# Autodesk Inventor assembly: fictief_zonnepaneel
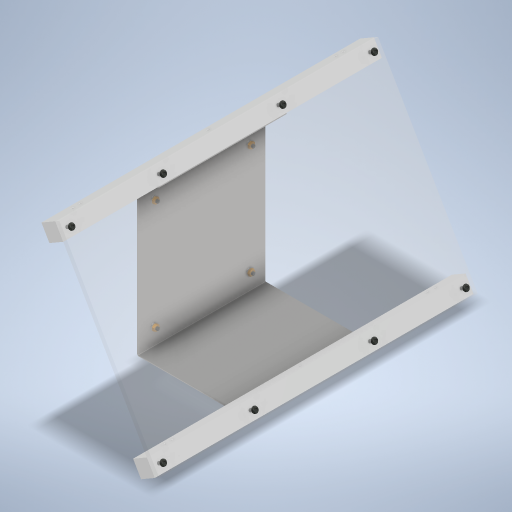
[picture p0: Inventor's stored thumbnail of the model, 512x512]
Saved by Autodesk Inventor 2023 (Build 270158000, 158)
## iProperties
Created: 2022-09-12
Part Number: fictief_zonnepaneel
Document SubType Name: Assembly
Designer: VoorL
Author: VoorL
## Documents named in this file (9)
- C:\Users\Ayoub\Documents\GitHub\zonnepaneel-concept\Opstelling_Zonnepaneel\fictief_zonnepaneel.iam
- C:\Users\Ayoub\Documents\GitHub\zonnepaneel-concept\Opstelling_Zonnepaneel\aluminium_stafmateriaal.ipt
- C:\Users\Ayoub\Documents\GitHub\zonnepaneel-concept\Opstelling_Zonnepaneel\Perspex_plaat.ipt
- C:\Users\Ayoub\Documents\GitHub\zonnepaneel-concept\Opstelling_Zonnepaneel\zetdeel_hoog.ipt
- C:\Users\Ayoub\Documents\GitHub\zonnepaneel-concept\Opstelling_Zonnepaneel\A4.ipt
- C:\Users\Ayoub\Documents\GitHub\zonnepaneel-concept\Opstelling_Zonnepaneel\rubberen_voetje.ipt
- C:\Users\Ayoub\Documents\GitHub\zonnepaneel-concept\Opstelling_Zonnepaneel\ISO 7380-1 - M4 x 10.ipt
- C:\Users\Ayoub\Documents\GitHub\zonnepaneel-concept\Opstelling_Zonnepaneel\DIN 125 - A 4,3.ipt
- C:\Users\Ayoub\Documents\GitHub\zonnepaneel-concept\Opstelling_Zonnepaneel\DIN EN ISO 4032 - M4.ipt
## Components (32 placed, 8 different names)
1. aluminium_stafmateriaal:1 — Mate:1, Mate:2, Mate:3
2. Perspex_plaat:1 — Mate:1, Mate:2, Mate:3, Mate:4, Mate:5, Mate:6, Mate:11, Flush:1, Flush:2, Insert:1, Insert:2, Insert:3, Insert:4, Insert:5, Insert:6, Insert:7, Insert:8
3. aluminium_stafmateriaal:2 — Mate:4, Mate:5, Mate:6, Mate:7, Mate:8, Mate:9
4. zetdeel_hoog:1 — Mate:7, Mate:8, Mate:9, Mate:10, Mate:12, Mate:13, Mate:14, Mate:15, Mate:16, Mate:17, Mate:18, Mate:19, Mate:26, Mate:27, Mate:29, Mate:31, Mate:32, Mate:33, Insert:10, Insert:11, Insert:12
5. A4:1 — Mate:11, Flush:1, Flush:2
6. rubberen_voetje:1 — Mate:12, Mate:16, Mate:20, Mate:21
7. rubberen_voetje:2 — Mate:15, Mate:19, Mate:24, Mate:25
8. rubberen_voetje:3 — Mate:13, Mate:17, Insert:9
9. rubberen_voetje:4 — Mate:14, Mate:18, Mate:22, Mate:23
10. ISO 7380-1 M4 x 10:1 — Insert:1
11. ISO 7380-1 M4 x 10:2 — Insert:2
12. ISO 7380-1 M4 x 10:3 — Insert:3
13. ISO 7380-1 M4 x 10:4 — Insert:4
14. ISO 7380-1 M4 x 10:5 — Insert:5
15. ISO 7380-1 M4 x 10:6 — Insert:6
16. ISO 7380-1 M4 x 10:7 — Insert:7
17. ISO 7380-1 M4 x 10:8 — Insert:8
18. ISO 7380-1 M4 x 10:9 — Insert:9, Mate:28, Mate:36
19. ISO 7380-1 M4 x 10:10 — Mate:20, Mate:21, Mate:34, Mate:41
20. ISO 7380-1 M4 x 10:11 — Mate:24, Mate:25, Mate:35, Mate:43
21. ISO 7380-1 M4 x 10:12 — Mate:22, Mate:23, Mate:30, Mate:38
22. DIN 125-1 A A 4,3:1 — Mate:28, Mate:29, Mate:37
23. DIN 125-1 A A 4,3:2 — Mate:32, Mate:35, Mate:42
24. DIN 125-1 A A 4,3:3 — Mate:33, Mate:34, Mate:40
25. DIN 125-1 A A 4,3:4 — Mate:30, Mate:31, Mate:39
26. DIN EN ISO 4032 M4:1 — Mate:36, Mate:37
27. DIN EN ISO 4032 M4:2 — Mate:38, Mate:39
28. DIN EN ISO 4032 M4:3 — Mate:40, Mate:41
29. DIN EN ISO 4032 M4:4 — Mate:42, Mate:43
30. ISO 7380-1 M4 x 10:13 — Insert:10
31. ISO 7380-1 M4 x 10:14 — Insert:11
32. ISO 7380-1 M4 x 10:15 — Insert:12
## Relationships (57: Mate 43, Insert 12, Flush 2)
- Mate:1: aluminium_stafmateriaal:1 ↔ Perspex_plaat:1
- Mate:2: aluminium_stafmateriaal:1 ↔ Perspex_plaat:1
- Mate:3: aluminium_stafmateriaal:1 ↔ Perspex_plaat:1
- Mate:4: Perspex_plaat:1 ↔ aluminium_stafmateriaal:2
- Mate:5: Perspex_plaat:1 ↔ aluminium_stafmateriaal:2
- Mate:6: Perspex_plaat:1 ↔ aluminium_stafmateriaal:2
- Mate:7: aluminium_stafmateriaal:2 ↔ zetdeel_hoog:1
- Mate:8: aluminium_stafmateriaal:2 ↔ zetdeel_hoog:1
- Mate:9: aluminium_stafmateriaal:2 ↔ zetdeel_hoog:1
- Mate:10: zetdeel_hoog:1
- Mate:11: Perspex_plaat:1 ↔ A4:1
- Flush:1 (50 mm): Perspex_plaat:1 ↔ A4:1
- Flush:2 (20 mm): Perspex_plaat:1 ↔ A4:1
- Mate:12: zetdeel_hoog:1 ↔ rubberen_voetje:1
- Mate:13: zetdeel_hoog:1 ↔ rubberen_voetje:3
- Mate:14: zetdeel_hoog:1 ↔ rubberen_voetje:4
- Mate:15: zetdeel_hoog:1 ↔ rubberen_voetje:2
- Mate:16: zetdeel_hoog:1 ↔ rubberen_voetje:1
- Mate:17: zetdeel_hoog:1 ↔ rubberen_voetje:3
- Mate:18: zetdeel_hoog:1 ↔ rubberen_voetje:4
- Mate:19: zetdeel_hoog:1 ↔ rubberen_voetje:2
- Insert:1: Perspex_plaat:1 ↔ ISO 7380-1 M4 x 10:1
- Insert:2: Perspex_plaat:1 ↔ ISO 7380-1 M4 x 10:2
- Insert:3: Perspex_plaat:1 ↔ ISO 7380-1 M4 x 10:3
- Insert:4: Perspex_plaat:1 ↔ ISO 7380-1 M4 x 10:4
- Insert:5: Perspex_plaat:1 ↔ ISO 7380-1 M4 x 10:5
- Insert:6: Perspex_plaat:1 ↔ ISO 7380-1 M4 x 10:6
- Insert:7: Perspex_plaat:1 ↔ ISO 7380-1 M4 x 10:7
- Insert:8: Perspex_plaat:1 ↔ ISO 7380-1 M4 x 10:8
- Insert:9: rubberen_voetje:3 ↔ ISO 7380-1 M4 x 10:9
- Mate:20: rubberen_voetje:1 ↔ ISO 7380-1 M4 x 10:10
- Mate:21: rubberen_voetje:1 ↔ ISO 7380-1 M4 x 10:10
- Mate:22: rubberen_voetje:4 ↔ ISO 7380-1 M4 x 10:12
- Mate:23: rubberen_voetje:4 ↔ ISO 7380-1 M4 x 10:12
- Mate:24: rubberen_voetje:2 ↔ ISO 7380-1 M4 x 10:11
- Mate:25: rubberen_voetje:2 ↔ ISO 7380-1 M4 x 10:11
- Mate:26: zetdeel_hoog:1
- Mate:27: zetdeel_hoog:1
- Mate:28: ISO 7380-1 M4 x 10:9 ↔ DIN 125-1 A A 4,3:1
- Mate:29: zetdeel_hoog:1 ↔ DIN 125-1 A A 4,3:1
- Mate:30: ISO 7380-1 M4 x 10:12 ↔ DIN 125-1 A A 4,3:4
- Mate:31: zetdeel_hoog:1 ↔ DIN 125-1 A A 4,3:4
- Mate:32: zetdeel_hoog:1 ↔ DIN 125-1 A A 4,3:2
- Mate:33: zetdeel_hoog:1 ↔ DIN 125-1 A A 4,3:3
- Mate:34: ISO 7380-1 M4 x 10:10 ↔ DIN 125-1 A A 4,3:3
- Mate:35: ISO 7380-1 M4 x 10:11 ↔ DIN 125-1 A A 4,3:2
- Mate:36: ISO 7380-1 M4 x 10:9 ↔ DIN EN ISO 4032 M4:1
- Mate:37: DIN 125-1 A A 4,3:1 ↔ DIN EN ISO 4032 M4:1
- Mate:38: ISO 7380-1 M4 x 10:12 ↔ DIN EN ISO 4032 M4:2
- Mate:39: DIN 125-1 A A 4,3:4 ↔ DIN EN ISO 4032 M4:2
- Mate:40: DIN 125-1 A A 4,3:3 ↔ DIN EN ISO 4032 M4:3
- Mate:41: ISO 7380-1 M4 x 10:10 ↔ DIN EN ISO 4032 M4:3
- Mate:42: DIN 125-1 A A 4,3:2 ↔ DIN EN ISO 4032 M4:4
- Mate:43: ISO 7380-1 M4 x 10:11 ↔ DIN EN ISO 4032 M4:4
- Insert:10: zetdeel_hoog:1 ↔ ISO 7380-1 M4 x 10:13
- Insert:11: zetdeel_hoog:1 ↔ ISO 7380-1 M4 x 10:14
- Insert:12: zetdeel_hoog:1 ↔ ISO 7380-1 M4 x 10:15
